# Autodesk Inventor assembly: 1002_Bias_Coil_MPSv2_v3
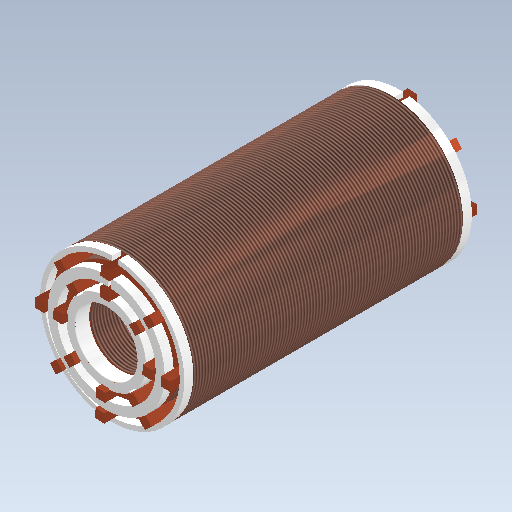
[picture p0: Inventor's stored thumbnail of the model, 512x512]
Saved by Autodesk Inventor 2021 (Build 250183000, 183)
## iProperties
Created: 2020-11-17
Part Number: 1002_Bias_Coil_MPSv2_v3
Document SubType Name: Assembly
Designer: Admin
Author: Admin
## Documents named in this file (8)
- C:\Users\Barksdale\Dropbox (MIT)\MPI Group Folder\MPS\MPSV2\1xxx Assemblies\10xx_Coil_Positioning_Assemblies\1002_Bias_Coil_MPSv2_v3.iam
- C:\Users\Barksdale\Dropbox (MIT)\MPI Group Folder\MPS\MPSV2\2xxx Coil Formers and Parts\22xx Bias Coil\4001_Bias_Coil_Holder_Tube_Mount_Base_MPSv2_v2.ipt
- C:\Users\Barksdale\Dropbox (MIT)\MPI Group Folder\MPS\MPSV2\2xxx Coil Formers and Parts\22xx Bias Coil\41xx_Bias_Coils\411x_Bias_Coil_Windings\4110_Bias_Coil_Layer1_MPSv2_v2.ipt
- C:\Users\Barksdale\Dropbox (MIT)\MPI Group Folder\MPS\MPSV2\2xxx Coil Formers and Parts\22xx Bias Coil\41xx_Bias_Coils\4100_Bias_Coil_Spacer_MPSv2_v2.ipt
- C:\Users\Barksdale\Dropbox (MIT)\MPI Group Folder\MPS\MPSV2\2xxx Coil Formers and Parts\22xx Bias Coil\41xx_Bias_Coils\411x_Bias_Coil_Windings\4111_Bias_Coil_Layer2_MPSv2_v2.ipt
- C:\Users\Barksdale\Dropbox (MIT)\MPI Group Folder\MPS\MPSV2\2xxx Coil Formers and Parts\22xx Bias Coil\4002_Bias_Coil_Holder_Tube_Mount_Layer2_MPSv2_v1.ipt
- C:\Users\Barksdale\Dropbox (MIT)\MPI Group Folder\MPS\MPSV2\2xxx Coil Formers and Parts\22xx Bias Coil\41xx_Bias_Coils\411x_Bias_Coil_Windings\4111_Bias_Coil_Layer3_MPSv2_v2.ipt
- C:\Users\Barksdale\Dropbox (MIT)\MPI Group Folder\MPS\MPSV2\2xxx Coil Formers and Parts\22xx Bias Coil\4002_Bias_Coil_Holder_Tube_Mount_Layer3_MPSv2_v2.ipt
## Components (25 placed, 7 different names)
1. 4001_Bias_Coil_Holder_Tube_Mount_Base_MPSv2_v2:1 — Mate:2, Mate:3, Angle:1, Angle:2, Flush:4
2. 4001_Bias_Coil_Holder_Tube_Mount_Base_MPSv2_v2:2 — Mate:1, Mate:4, Angle:2, Flush:1, Mate:5, Flush:3, Mate:10
3. 4110_Bias_Coil_Layer1_MPSv2_v2:1 — Mate:1, Mate:2, Mate:3, Mate:4, Tangent:1, Mate:6, Flush:2, Mate:9
4. 4111_Bias_Coil_Layer2_MPSv2_v2:1 — Mate:6, Flush:2, Mate:7, Mate:8, Flush:7
5. 4002_Bias_Coil_Holder_Tube_Mount_Layer2_MPSv2_v1:2 — Mate:7, Flush:3, Tangent:2
6. 4002_Bias_Coil_Holder_Tube_Mount_Layer2_MPSv2_v1:1 — Mate:8, Flush:4
7. 4111_Bias_Coil_Layer3_MPSv2_v2:1 — Mate:9, Flush:7, Mate:11, Mate:12, Mate:13
8. 4002_Bias_Coil_Holder_Tube_Mount_Layer3_MPSv2_v2:1 — Mate:10, Mate:11
9. 4002_Bias_Coil_Holder_Tube_Mount_Layer3_MPSv2_v2:2 — Mate:12, Mate:13
10. 4100_Bias_Coil_Spacer_MPSv2_v2:1 — Angle:1, Tangent:1, Flush:1, Mate:5
11. 4100_Bias_Coil_Spacer_MPSv2_v2:2 — Flush:5, Angle:3, Flush:6
12. 4100_Bias_Coil_Spacer_MPSv2_v2:3
13. 4100_Bias_Coil_Spacer_MPSv2_v2:4
14. 4100_Bias_Coil_Spacer_MPSv2_v2:5
15. 4100_Bias_Coil_Spacer_MPSv2_v2:6
16. 4100_Bias_Coil_Spacer_MPSv2_v2:7
17. 4100_Bias_Coil_Spacer_MPSv2_v2:8
18. 4100_Bias_Coil_Spacer_MPSv2_v2:9 — Flush:5, Angle:3, Tangent:2, Flush:6
19. 4100_Bias_Coil_Spacer_MPSv2_v2:10
20. 4100_Bias_Coil_Spacer_MPSv2_v2:11
21. 4100_Bias_Coil_Spacer_MPSv2_v2:12
22. 4100_Bias_Coil_Spacer_MPSv2_v2:13
23. 4100_Bias_Coil_Spacer_MPSv2_v2:14
24. 4100_Bias_Coil_Spacer_MPSv2_v2:15
25. 4100_Bias_Coil_Spacer_MPSv2_v2:16
## Component patterns: (8 elements, first: 4100_Bias_Coil_Spacer_MPSv2_v2:1), (8 elements, first: 4100_Bias_Coil_Spacer_MPSv2_v2:9)
## Relationships (25: Mate 13, Flush 7, Angle 3, Tangent 2)
- Mate:1: 4001_Bias_Coil_Holder_Tube_Mount_Base_MPSv2_v2:2 ↔ 4110_Bias_Coil_Layer1_MPSv2_v2:1
- Mate:2: 4001_Bias_Coil_Holder_Tube_Mount_Base_MPSv2_v2:1 ↔ 4110_Bias_Coil_Layer1_MPSv2_v2:1
- Mate:3: 4001_Bias_Coil_Holder_Tube_Mount_Base_MPSv2_v2:1 ↔ 4110_Bias_Coil_Layer1_MPSv2_v2:1
- Mate:4: 4001_Bias_Coil_Holder_Tube_Mount_Base_MPSv2_v2:2 ↔ 4110_Bias_Coil_Layer1_MPSv2_v2:1
- Angle:1 (0 deg): 4001_Bias_Coil_Holder_Tube_Mount_Base_MPSv2_v2:1 ↔ 4100_Bias_Coil_Spacer_MPSv2_v2:1
- Angle:2 (0 deg): 4001_Bias_Coil_Holder_Tube_Mount_Base_MPSv2_v2:1 ↔ 4001_Bias_Coil_Holder_Tube_Mount_Base_MPSv2_v2:2
- Tangent:1: 4110_Bias_Coil_Layer1_MPSv2_v2:1 ↔ 4100_Bias_Coil_Spacer_MPSv2_v2:1
- Flush:1 (-2.5 mm): 4001_Bias_Coil_Holder_Tube_Mount_Base_MPSv2_v2:2 ↔ 4100_Bias_Coil_Spacer_MPSv2_v2:1
- Mate:5 (-0.5 mm): 4001_Bias_Coil_Holder_Tube_Mount_Base_MPSv2_v2:2 ↔ 4100_Bias_Coil_Spacer_MPSv2_v2:1
- Mate:6: 4110_Bias_Coil_Layer1_MPSv2_v2:1 ↔ 4111_Bias_Coil_Layer2_MPSv2_v2:1
- Flush:2: 4110_Bias_Coil_Layer1_MPSv2_v2:1 ↔ 4111_Bias_Coil_Layer2_MPSv2_v2:1
- Mate:7: 4111_Bias_Coil_Layer2_MPSv2_v2:1 ↔ 4002_Bias_Coil_Holder_Tube_Mount_Layer2_MPSv2_v1:2
- Mate:8: 4111_Bias_Coil_Layer2_MPSv2_v2:1 ↔ 4002_Bias_Coil_Holder_Tube_Mount_Layer2_MPSv2_v1:1
- Flush:3: 4001_Bias_Coil_Holder_Tube_Mount_Base_MPSv2_v2:2 ↔ 4002_Bias_Coil_Holder_Tube_Mount_Layer2_MPSv2_v1:2
- Flush:4: 4001_Bias_Coil_Holder_Tube_Mount_Base_MPSv2_v2:1 ↔ 4002_Bias_Coil_Holder_Tube_Mount_Layer2_MPSv2_v1:1
- Flush:5: 4100_Bias_Coil_Spacer_MPSv2_v2:2 ↔ 4100_Bias_Coil_Spacer_MPSv2_v2:9
- Angle:3 (0 deg): 4100_Bias_Coil_Spacer_MPSv2_v2:2 ↔ 4100_Bias_Coil_Spacer_MPSv2_v2:9
- Tangent:2: 4002_Bias_Coil_Holder_Tube_Mount_Layer2_MPSv2_v1:2 ↔ 4100_Bias_Coil_Spacer_MPSv2_v2:9
- Flush:6: 4100_Bias_Coil_Spacer_MPSv2_v2:2 ↔ 4100_Bias_Coil_Spacer_MPSv2_v2:9
- Mate:9: 4110_Bias_Coil_Layer1_MPSv2_v2:1 ↔ 4111_Bias_Coil_Layer3_MPSv2_v2:1
- Flush:7: 4111_Bias_Coil_Layer2_MPSv2_v2:1 ↔ 4111_Bias_Coil_Layer3_MPSv2_v2:1
- Mate:10: 4001_Bias_Coil_Holder_Tube_Mount_Base_MPSv2_v2:2 ↔ 4002_Bias_Coil_Holder_Tube_Mount_Layer3_MPSv2_v2:1
- Mate:11: 4111_Bias_Coil_Layer3_MPSv2_v2:1 ↔ 4002_Bias_Coil_Holder_Tube_Mount_Layer3_MPSv2_v2:1
- Mate:12: 4111_Bias_Coil_Layer3_MPSv2_v2:1 ↔ 4002_Bias_Coil_Holder_Tube_Mount_Layer3_MPSv2_v2:2
- Mate:13: 4111_Bias_Coil_Layer3_MPSv2_v2:1 ↔ 4002_Bias_Coil_Holder_Tube_Mount_Layer3_MPSv2_v2:2
